# Autodesk Inventor assembly: 3d model final
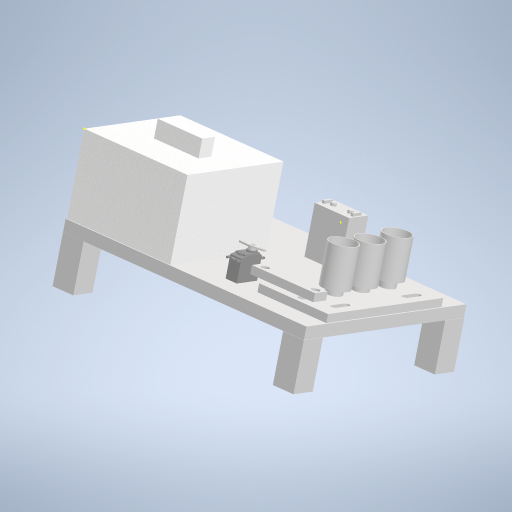
[picture p0: Inventor's stored thumbnail of the model, 512x512]
Saved by Autodesk Inventor 2023 (Build 270158000, 158)
## iProperties
Created: 2022-06-23
Part Number: 3d model final
Document SubType Name: Assembly
Designer: Shivan
Author: Shivan
## Documents named in this file (10)
- C:\Users\Shivan\Desktop\3D models\3d model final.iam
- C:\Users\Shivan\Desktop\3D models\stand.ipt
- C:\Users\Shivan\Desktop\3D models\Sliding Plate.ipt
- C:\Users\Shivan\Desktop\3D models\expo arm.ipt
- C:\Users\Shivan\Desktop\3D models\Main base.ipt
- C:\Users\Shivan\Desktop\3D models\battery.ipt
- C:\Users\Shivan\Desktop\3D models\Servo motor.ipt
- C:\Users\Shivan\Desktop\3D models\Servo arm.ipt
- C:\Users\Shivan\Desktop\3D models\water tank 1.ipt
- C:\Users\Shivan\Desktop\3D models\new seed container.ipt
## Components (14 placed, 9 different names)
1. stand:1 — Mate:9
2. stand:2 — Mate:7
3. stand:3 — Mate:10
4. stand:4 — Mate:8
5. Sliding Plate:1 — Mate:6, Mate:11, Mate:12, Mate:16, Mate:17, Mate:18
6. expo arm:1 — Mate:6, Mate:12
7. Main base:1 — Mate:7, Mate:8, Mate:9, Mate:10, Mate:11, Mate:13, Mate:14, Mate:19
8. battery:1 — Mate:13
9. Servo motor:1 — Mate:14, Mate:15
10. Servo arm:1 — Mate:15
11. water tank 1:1 — Mate:19
12. new seed container:1 — Mate:16
13. new seed container:2 — Mate:18
14. new seed container:3 — Mate:17
## Relationships (14: Mate 14)
- Mate:6: Sliding Plate:1 ↔ expo arm:1
- Mate:7: stand:2 ↔ Main base:1
- Mate:8: stand:4 ↔ Main base:1
- Mate:9: stand:1 ↔ Main base:1
- Mate:10: stand:3 ↔ Main base:1
- Mate:11: Sliding Plate:1 ↔ Main base:1
- Mate:12: Sliding Plate:1 ↔ expo arm:1
- Mate:13: Main base:1 ↔ battery:1
- Mate:14: Main base:1 ↔ Servo motor:1
- Mate:15: Servo motor:1 ↔ Servo arm:1
- Mate:16: Sliding Plate:1 ↔ new seed container:1
- Mate:17: Sliding Plate:1 ↔ new seed container:3
- Mate:18: Sliding Plate:1 ↔ new seed container:2
- Mate:19: Main base:1 ↔ water tank 1:1
